# Autodesk Inventor assembly: 8020ChassisSupport
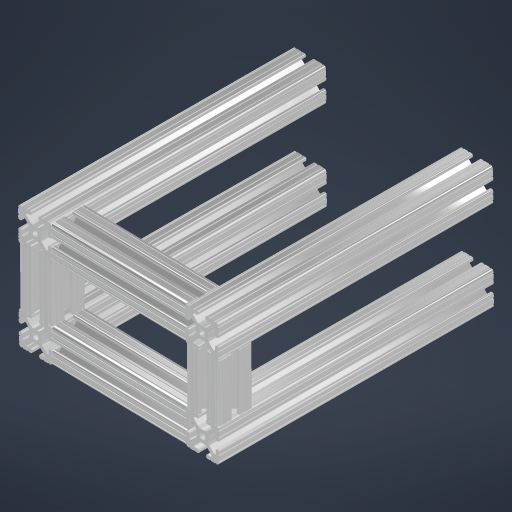
[picture p0: Inventor's stored thumbnail of the model, 512x512]
Saved by Autodesk Inventor 2023 (Build 270158000, 158)
## iProperties
Created: 2022-04-12
Part Number: 8020ChassisSupport
Document SubType Name: Assembly
Designer: Nebil Oumer
Author: Nebil Oumer
## Documents named in this file (4)
- E:\SBRT\testRoboRescue\Chassis\Frame\8020ChassisSupport.iam
- E:\SBRT\testRoboRescue\Chassis\Frame\8020Support_Width.ipt
- E:\SBRT\testRoboRescue\Chassis\Frame\8020Support_Length.ipt
- E:\SBRT\testRoboRescue\Chassis\Frame\8020Support_height.ipt
## Components (8 placed, 3 different names)
1. 8020Support_Width:1 — Mate:3, Flush:5, Flush:6, Flush:7, Flush:8, Mate:4, Flush:14
2. 8020Support_Width:2 — Mate:1, Flush:1, Flush:2, Mate:2, Flush:3, Flush:4
3. 8020Support_Length:1 — Mate:3, Flush:5, Flush:6
4. 8020Support_Length:2 — Mate:2, Flush:3, Flush:4, Mate:6, Flush:11, Flush:12
5. 8020Support_Length:3 — Mate:1, Flush:1, Flush:2, Mate:5, Flush:9, Flush:10
6. 8020Support_Length:4 — Flush:7, Flush:8, Mate:4, Mate:7, Flush:13
7. 8020Support_height:1 — Mate:5, Flush:9, Flush:10
8. 8020Support_height:2 — Mate:6, Flush:11, Flush:12, Mate:7, Flush:13, Flush:14
## Relationships (21: Flush 14, Mate 7)
- Mate:1: 8020Support_Width:2 ↔ 8020Support_Length:3
- Flush:1: 8020Support_Width:2 ↔ 8020Support_Length:3
- Flush:2: 8020Support_Width:2 ↔ 8020Support_Length:3
- Mate:2: 8020Support_Width:2 ↔ 8020Support_Length:2
- Flush:3: 8020Support_Width:2 ↔ 8020Support_Length:2
- Flush:4: 8020Support_Width:2 ↔ 8020Support_Length:2
- Mate:3: 8020Support_Width:1 ↔ 8020Support_Length:1
- Flush:5: 8020Support_Width:1 ↔ 8020Support_Length:1
- Flush:6: 8020Support_Width:1 ↔ 8020Support_Length:1
- Flush:7: 8020Support_Width:1 ↔ 8020Support_Length:4
- Flush:8: 8020Support_Width:1 ↔ 8020Support_Length:4
- Mate:4: 8020Support_Width:1 ↔ 8020Support_Length:4
- Mate:5: 8020Support_Length:3 ↔ 8020Support_height:1
- Flush:9: 8020Support_Length:3 ↔ 8020Support_height:1
- Flush:10: 8020Support_Length:3 ↔ 8020Support_height:1
- Mate:6: 8020Support_Length:2 ↔ 8020Support_height:2
- Flush:11: 8020Support_Length:2 ↔ 8020Support_height:2
- Flush:12: 8020Support_Length:2 ↔ 8020Support_height:2
- Mate:7: 8020Support_Length:4 ↔ 8020Support_height:2
- Flush:13: 8020Support_Length:4 ↔ 8020Support_height:2
- Flush:14: 8020Support_Width:1 ↔ 8020Support_height:2
